# Autodesk Inventor assembly: Track Design 9-3-19
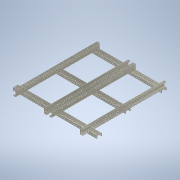
[picture p0: Inventor's stored thumbnail of the model, 180x180]
Saved by Autodesk Inventor 2020 (Build 240168000, 168)
## iProperties
Created: 2019-07-25
Part Number: Track Design 9-3-19
Document SubType Name: Assembly
Designer: Corey
Author: Corey
## Documents named in this file (3)
- C:\Users\Corey\Documents\Tower-Takeover-CAD\Track Design 9-3-19.iam
- C:\Users\Corey\Documents\Tower-Takeover-CAD\Parts\Structure\C-Channels\Aluminum\2-Wide\Aluminum C-Channel 1x2x1x35.ipt
- C:\Users\Corey\Documents\Tower-Takeover-CAD\Parts\Structure\C-Channels\Aluminum\2-Wide\Aluminum C-Channel 1x2x1x29.ipt
## Components (7 placed, 2 different names)
1. Aluminum C-Channel 1x2x1x35:1 — Mate:2, Mate:3, Mate:4, Flush:3, Flush:5, Flush:7, Mate:6, Flush:13, Flush:14, Flush:15, Flush:16, Flush:19
2. Aluminum C-Channel 1x2x1x35:2 — Mate:2, Flush:5, Flush:16
3. Aluminum C-Channel 1x2x1x35:3 — Mate:6, Flush:13, Flush:14
4. Aluminum C-Channel 1x2x1x35:4 — Mate:3, Flush:3, Flush:15
5. Aluminum C-Channel 1x2x1x35:5 — Mate:4, Flush:7, Flush:19, Mate:7, Flush:20, Flush:21, Mate:8, Flush:22, Flush:23
6. Aluminum C-Channel 1x2x1x29:1 — Mate:8, Flush:22, Flush:23
7. Aluminum C-Channel 1x2x1x29:2 — Mate:7, Flush:20, Flush:21
## Relationships (18: Flush 12, Mate 6)
- Mate:2: Aluminum C-Channel 1x2x1x35:1 ↔ Aluminum C-Channel 1x2x1x35:2
- Mate:3: Aluminum C-Channel 1x2x1x35:1 ↔ Aluminum C-Channel 1x2x1x35:4
- Mate:4: Aluminum C-Channel 1x2x1x35:1 ↔ Aluminum C-Channel 1x2x1x35:5
- Flush:3: Aluminum C-Channel 1x2x1x35:1 ↔ Aluminum C-Channel 1x2x1x35:4
- Flush:5: Aluminum C-Channel 1x2x1x35:1 ↔ Aluminum C-Channel 1x2x1x35:2
- Flush:7: Aluminum C-Channel 1x2x1x35:1 ↔ Aluminum C-Channel 1x2x1x35:5
- Mate:6: Aluminum C-Channel 1x2x1x35:1 ↔ Aluminum C-Channel 1x2x1x35:3
- Flush:13: Aluminum C-Channel 1x2x1x35:1 ↔ Aluminum C-Channel 1x2x1x35:3
- Flush:14: Aluminum C-Channel 1x2x1x35:1 ↔ Aluminum C-Channel 1x2x1x35:3
- Flush:15: Aluminum C-Channel 1x2x1x35:1 ↔ Aluminum C-Channel 1x2x1x35:4
- Flush:16: Aluminum C-Channel 1x2x1x35:1 ↔ Aluminum C-Channel 1x2x1x35:2
- Flush:19: Aluminum C-Channel 1x2x1x35:1 ↔ Aluminum C-Channel 1x2x1x35:5
- Mate:7: Aluminum C-Channel 1x2x1x35:5 ↔ Aluminum C-Channel 1x2x1x29:2
- Flush:20: Aluminum C-Channel 1x2x1x35:5 ↔ Aluminum C-Channel 1x2x1x29:2
- Flush:21: Aluminum C-Channel 1x2x1x35:5 ↔ Aluminum C-Channel 1x2x1x29:2
- Mate:8: Aluminum C-Channel 1x2x1x35:5 ↔ Aluminum C-Channel 1x2x1x29:1
- Flush:22: Aluminum C-Channel 1x2x1x35:5 ↔ Aluminum C-Channel 1x2x1x29:1
- Flush:23: Aluminum C-Channel 1x2x1x35:5 ↔ Aluminum C-Channel 1x2x1x29:1
